# Autodesk Inventor assembly: ABME-2020-4-L
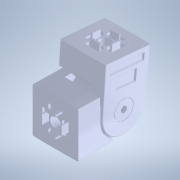
[picture p0: Inventor's stored thumbnail of the model, 180x180]
Saved by Autodesk Inventor 2021.1 (Build 251245010, 245A)
## iProperties
Created: 2018-09-13
Part Number: ABME-2020-4-L
Description: STEP AP214
Document SubType Name: Assembly
Designer: gisen
Sending System: SolidWorks 2018
Preprocessor: SwSTEP 2.0
Title: ABME-2020-4-L.STEP
Revision Number: ANY
## Documents named in this file (5)
- C:\Users\gisen\GitProjects\CAD-Data\GeneralComponentsTemplate\Fittings\BasicFrameMultiEndConnectorL.iam
- C:\Users\gisen\GitProjects\CAD-Data\GeneralComponentsTemplate\Fittings\BasicFrameMultiEndConnectorL\ABME-2020-4-L.ipt
- C:\Users\gisen\GitProjects\CAD-Data\GeneralComponentsTemplate\Fittings\BasicFrameMultiEndConnectorL\ABME-2020-4-L-2.ipt
- C:\Users\gisen\GitProjects\CAD-Data\GeneralComponentsTemplate\Fittings\BasicFrameMultiEndConnectorL\ABME-2020-4-L-1.ipt
- C:\Users\gisen\GitProjects\CAD-Data\GeneralComponentsTemplate\Fittings\BasicFrameMultiEndConnectorL\ABME-2020-4-L-3.ipt
## Components (7 placed, 7 different names)
1. ABME-2020-4-L_1 — メイト:6, フラッシュ:2, メイト:7, メイト:8, メイト:9
2. RlN^²_2 — メイト:1, メイト:2, メイト:3, メイト:4, メイト:5, メイト:7, メイト:8
3. J[_3 — メイト:1, メイト:2
4. J[_4 — メイト:6
5. ABME-2020-4-L_5 — メイト:4, メイト:5, フラッシュ:1
6. FCS-04_ÃÞÌ«ÙÄ L8_8 — フラッシュ:2, メイト:9
7. FCS-04_ÃÞÌ«ÙÄ L8_9 — メイト:3, フラッシュ:1
## Relationships (11: Mate 9, Flush 2)
- メイト:1 [Mate]: RlN^²_2 ↔ J[_3
- メイト:2 [Mate]: RlN^²_2 ↔ J[_3
- メイト:3 [Mate]: RlN^²_2 ↔ FCS-04_ÃÞÌ«ÙÄ L8_9
- メイト:4 [Mate]: RlN^²_2 ↔ ABME-2020-4-L_5
- メイト:5 [Mate]: RlN^²_2 ↔ ABME-2020-4-L_5
- フラッシュ:1 [Flush]: ABME-2020-4-L_5 ↔ FCS-04_ÃÞÌ«ÙÄ L8_9
- メイト:6 [Mate]: ABME-2020-4-L_1 ↔ J[_4
- フラッシュ:2 [Flush]: ABME-2020-4-L_1 ↔ FCS-04_ÃÞÌ«ÙÄ L8_8
- メイト:7 [Mate]: ABME-2020-4-L_1 ↔ RlN^²_2
- メイト:8 [Mate]: ABME-2020-4-L_1 ↔ RlN^²_2
- メイト:9 [Mate]: ABME-2020-4-L_1 ↔ FCS-04_ÃÞÌ«ÙÄ L8_8
